# Autodesk Inventor assembly: Servo
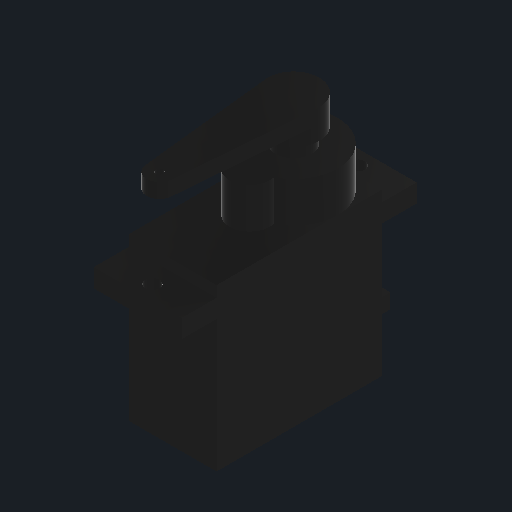
[picture p0: Inventor's stored thumbnail of the model, 512x512]
Saved by Autodesk Inventor 2024 (Build 280153000, 153)
## iProperties
Created: 2025-01-02
Part Number: Servo
Document SubType Name: Assembly
Designer: huj31
Author: huj31
## Documents named in this file (3)
- C:\Users\huj31\OneDrive\Documents\__ school\Capstone\CAD\Servo.iam
- C:\Users\huj31\OneDrive\Documents\__ school\Capstone\CAD\servo.ipt
- C:\Users\huj31\OneDrive\Documents\__ school\Capstone\CAD\servohorn.ipt
## Components (2 placed, 2 different names)
1. servo:1 — Mate:1, Mate:2
2. servohorn:1 — Mate:1, Mate:2
## Relationships (2: Mate 2)
- Mate:1: servo:1 ↔ servohorn:1
- Mate:2: servo:1 ↔ servohorn:1
